# Autodesk Inventor assembly: Ensamble motor
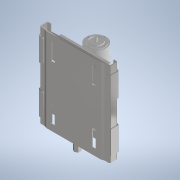
[picture p0: Inventor's stored thumbnail of the model, 180x180]
Saved by Autodesk Inventor 2022.2 (Build 262287000, 287)
## iProperties
Created: 2022-02-10
Part Number: Ensamble motor
Document SubType Name: Assembly
Designer: USUARIO
Author: USUARIO
## Documents named in this file (4)
- C:\Users\USUARIO\Downloads\Proyecto diseño\Ensamble motor.iam
- C:\Users\USUARIO\Downloads\Proyecto diseño\Slitta SMA340 - 90\132N.ipt
- C:\Users\USUARIO\Downloads\Proyecto diseño\Base motor.ipt
- C:\Users\USUARIO\Downloads\Proyecto diseño\Motor.ipt
## Components (2 placed, 2 different names)
1. 132N:1 — Coincidencia:1, Nivelación:1
2. Motor:1 — Coincidencia:1, Nivelación:1
## Relationships (2: Mate 1, Flush 1)
- Coincidencia:1 [Mate]: 132N:1 ↔ Motor:1
- Nivelación:1 [Flush]: 132N:1 ↔ Motor:1
